# Autodesk Inventor assembly: МД.001.700 - Поворотный механизм
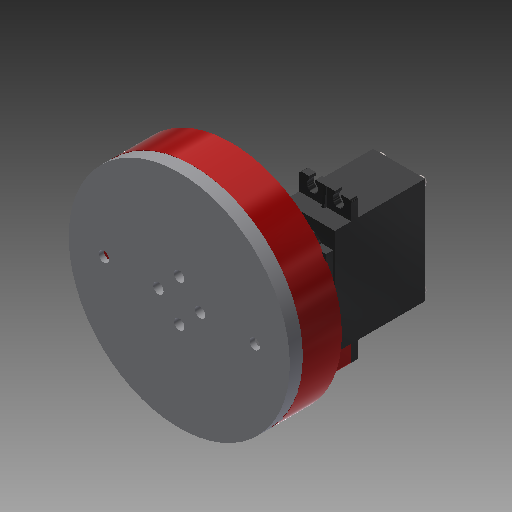
[picture p0: Inventor's stored thumbnail of the model, 512x512]
Saved by Autodesk Inventor 2019 (Build 230136000, 136)
## iProperties
Created: 2019-12-29
Part Number: МД.001.700 - Поворотный механизм
Material: Типовые
Document SubType Name: Assembly
Designer: Петров Иван
Author: Петров Иван
## Documents named in this file (6)
- E:\IVAN\Ivan_desktop\GitHub\Arm_manip\hardware\МД.001.700 - Поворотный механизм.iam
- E:\IVAN\Ivan_desktop\GitHub\Arm_manip\hardware\МД.001.701 - Опора.ipt
- E:\IVAN\Ivan_desktop\GitHub\Arm_manip\hardware\МД.001.700_1 - Редуктор поворотного механизма.iam
- E:\IVAN\Ivan_desktop\GitHub\Arm_manip\hardware\Standart_things\tower prone.ipt
- E:\IVAN\Ivan_desktop\GitHub\Arm_manip\hardware\Standart_things\Potentiometer.ipt
- E:\IVAN\Ivan_desktop\GitHub\Arm_manip\hardware\МД.001.702 - Крышка.ipt
## Components (5 placed, 5 different names)
1. МД.001.701 - Опора:1 — Совмещение:1, Совмещение:2, Совмещение:3, Совмещение:6, Совмещение:7, Совмещение:8, Совмещение:9, Совмещение:11, Совмещение:12
2. Цилиндрическое зубчатое зацепление:1 [sub-assembly] — Совмещение:4, Совмещение:5, Совмещение:9
3. tower prone:1 — Совмещение:1, Совмещение:2, Совмещение:3, Совмещение:4, Совмещение:5
4. Potentiometer:1 — Совмещение:6, Совмещение:7, Совмещение:8
5. МД.001.702 - Крышка:1 — Совмещение:11, Совмещение:12
## Relationships (11: Mate 11)
- Совмещение:1 [Mate]: МД.001.701 - Опора:1 ↔ tower prone:1
- Совмещение:2 [Mate]: МД.001.701 - Опора:1 ↔ tower prone:1
- Совмещение:3 [Mate]: МД.001.701 - Опора:1 ↔ tower prone:1
- Совмещение:4 [Mate]: Цилиндрическое зубчатое зацепление:1 ↔ tower prone:1
- Совмещение:5 [Mate]: Цилиндрическое зубчатое зацепление:1 ↔ tower prone:1
- Совмещение:6 [Mate]: МД.001.701 - Опора:1 ↔ Potentiometer:1
- Совмещение:7 [Mate]: МД.001.701 - Опора:1 ↔ Potentiometer:1
- Совмещение:8 [Mate]: МД.001.701 - Опора:1 ↔ Potentiometer:1
- Совмещение:9 [Mate]: МД.001.701 - Опора:1 ↔ Цилиндрическое зубчатое зацепление:1
- Совмещение:11 [Mate]: МД.001.701 - Опора:1 ↔ МД.001.702 - Крышка:1
- Совмещение:12 [Mate]: МД.001.701 - Опора:1 ↔ МД.001.702 - Крышка:1
